# Autodesk Inventor assembly: gripper
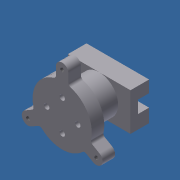
[picture p0: Inventor's stored thumbnail of the model, 180x180]
Saved by Autodesk Inventor 2012 (Build 160160000, 160)
## iProperties
Created: 2012-07-09
Part Number: gripper
Document SubType Name: Assembly
Designer: Ed
Author: Ed
## Documents named in this file (4)
- C:\Users\Edward\Documents\masters\CAD\Gripper\gripper.iam
- C:\Users\Edward\Documents\masters\CAD\Gripper\gripper plate.ipt
- C:\Users\Edward\Documents\masters\CAD\Gripper\gripper.ipt
- C:\Users\Edward\Documents\masters\CAD\Gripper\IRB120 plate.ipt
## Components (3 placed, 3 different names)
1. gripper plate:1 — Insert:1, Insert:2, Insert:3, Insert:4
2. gripper:1 — Insert:1, Insert:4
3. IRB120 plate:1 — Insert:2, Insert:3
## Relationships (4: Insert 4)
- Insert:1: gripper plate:1 ↔ gripper:1
- Insert:2: gripper plate:1 ↔ IRB120 plate:1
- Insert:3: gripper plate:1 ↔ IRB120 plate:1
- Insert:4: gripper plate:1 ↔ gripper:1
